# Autodesk Inventor assembly: Assembly
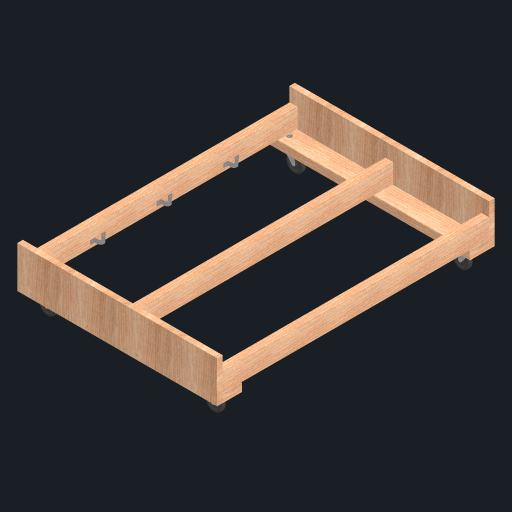
[picture p0: Inventor's stored thumbnail of the model, 512x512]
Saved by Autodesk Inventor 2024.2 (Build 282272000, 272)
## iProperties
Created: 2025-06-28
Part Number: Assembly
Document SubType Name: Assembly
Designer: Bryan
Mass: 15499.4 g
Surface Area: 23116.4 cm^2
Volume: 27379.6 cm^3
Density: 0.566091 g/cm^3
Author: Bryan
## Documents named in this file (14)
- C:\Users\bobsb\OneDrive\Documents\GitHub\PlateRack_Robotics\Assembly.iam
- C:\Users\bobsb\OneDrive\Documents\GitHub\PlateRack_Robotics\2834T25_Threaded-Stem Swivel Caster.ipt
- C:\Users\bobsb\OneDrive\Documents\GitHub\PlateRack_Robotics\Horizontal Beam 3ft.ipt
- C:\Users\bobsb\OneDrive\Documents\GitHub\PlateRack_Robotics\Horizontal Beam 4ft.ipt
- C:\Users\bobsb\OneDrive\Documents\GitHub\PlateRack_Robotics\91903A032_Medium-Strength Steel Extra-Wide Hex Nut.ipt
- C:\Users\bobsb\OneDrive\Documents\GitHub\PlateRack_Robotics\Side Panel.ipt
- C:\Users\bobsb\OneDrive\Documents\GitHub\PlateRack_Robotics\9439T44_Routing Clamp.ipt
- C:\Users\bobsb\OneDrive\Documents\GitHub\PlateRack_Robotics\90031A580_Phillips Flat Head Screws for Wood.ipt
- C:\Users\bobsb\OneDrive\Documents\GitHub\PlateRack_Robotics\Assembly\AIP\FEA\f3xuib2qo.fins
- C:\Users\bobsb\OneDrive\Documents\GitHub\PlateRack_Robotics\Assembly\AIP\FEA\f3xuib2qo.fsat
- C:\Users\bobsb\OneDrive\Documents\GitHub\PlateRack_Robotics\Assembly\AIP\FEA\f3xuib2qo.ftes
- C:\Users\bobsb\OneDrive\Documents\GitHub\PlateRack_Robotics\Assembly\AIP\FEA\f3xuib2qo.fwiz
- C:\Users\bobsb\OneDrive\Documents\GitHub\PlateRack_Robotics\Assembly\AIP\FEA\f3xuib2w0.fmsh
- C:\Users\bobsb\OneDrive\Documents\GitHub\PlateRack_Robotics\Assembly\AIP\FEA\f3xuib2w1.fres
## Components (77 placed, 7 different names)
1. 2834T25_Threaded-Stem Swivel Caster:1 — Mate:1, Mate:2, Angle:1, Mate:6
2. Horizontal Beam 3ft:1 — Mate:1, Mate:2, Angle:1, Mate:3, Mate:4, Angle:2, Flush:1, Mate:5, Flush:2, Mate:7, Mate:8, Mate:9, Flush:3, Flush:4, Flush:5, Mate:12, Mate:22, Flush:8, Mate:55, Flush:25, Mate:56, Flush:26, Mate:57, Flush:27
3. Horizontal Beam 4ft:1 — Flush:1, Mate:5, Flush:2, Mate:10, Flush:6, Flush:7, Flush:9, Flush:11, Mate:33, Mate:34, Mate:35, Mate:36, Mate:37, Mate:38, Mate:39, Mate:40, Mate:41
4. 2834T25_Threaded-Stem Swivel Caster:2 — Mate:3, Mate:4, Angle:2, Mate:11
5. 91903A032_Medium-Strength Steel Extra-Wide Hex Nut:1 — Mate:6, Mate:7
6. Horizontal Beam 4ft:2 — Mate:9, Flush:3, Flush:4, Mate:24, Mate:25, Mate:26, Mate:27, Mate:28, Mate:29, Mate:30, Mate:31, Mate:32
7. Horizontal Beam 4ft:3 — Mate:8, Flush:5, Mate:10, Mate:21
8. 91903A032_Medium-Strength Steel Extra-Wide Hex Nut:2 — Mate:11, Mate:12
9. 2834T25_Threaded-Stem Swivel Caster:3
10. Horizontal Beam 3ft:2 — Mate:21, Flush:6, Flush:7, Flush:10, Mate:23, Mate:52, Flush:22, Mate:53, Flush:23, Mate:54, Flush:24
11. 2834T25_Threaded-Stem Swivel Caster:4
12. 91903A032_Medium-Strength Steel Extra-Wide Hex Nut:3
13. 91903A032_Medium-Strength Steel Extra-Wide Hex Nut:4
14. Side Panel:1 — Mate:22, Flush:8, Flush:9, Mate:42, Flush:12, Mate:43, Flush:13, Mate:44, Flush:14, Mate:45, Flush:15, Mate:46, Flush:16
15. Side Panel:2 — Flush:10, Flush:11, Mate:23, Mate:47, Flush:17, Mate:48, Flush:18, Mate:49, Flush:19, Mate:50, Flush:20, Mate:51, Flush:21
16. 9439T44_Routing Clamp:1 — Mate:24, Mate:25, Mate:26
17. 9439T44_Routing Clamp:2 — Mate:27, Mate:28, Mate:29
18. 9439T44_Routing Clamp:3 — Mate:30, Mate:31, Mate:32
19. 9439T44_Routing Clamp:4 — Mate:33, Mate:40, Mate:41
20. 9439T44_Routing Clamp:5 — Mate:34, Mate:38, Mate:39
21. 9439T44_Routing Clamp:6 — Mate:35, Mate:36, Mate:37
22. 90031A580_Phillips Flat Head Screws for Wood:1 — Mate:42, Flush:12
23. 90031A580_Phillips Flat Head Screws for Wood:18 — Mate:45, Flush:15
24. 90031A580_Phillips Flat Head Screws for Wood:19 — Mate:46, Flush:16
25. 90031A580_Phillips Flat Head Screws for Wood:20 — Mate:47, Flush:17
26. 90031A580_Phillips Flat Head Screws for Wood:21 — Mate:48, Flush:18
27. 90031A580_Phillips Flat Head Screws for Wood:22 — Mate:49, Flush:19
28. 90031A580_Phillips Flat Head Screws for Wood:2 — Mate:43, Flush:13
29. 90031A580_Phillips Flat Head Screws for Wood:3
30. 90031A580_Phillips Flat Head Screws for Wood:4
31. 90031A580_Phillips Flat Head Screws for Wood:5
32. 90031A580_Phillips Flat Head Screws for Wood:6
33. 90031A580_Phillips Flat Head Screws for Wood:7
34. 90031A580_Phillips Flat Head Screws for Wood:8
35. 90031A580_Phillips Flat Head Screws for Wood:9
36. 90031A580_Phillips Flat Head Screws for Wood:10 — Mate:44, Flush:14
37. 90031A580_Phillips Flat Head Screws for Wood:11
38. 90031A580_Phillips Flat Head Screws for Wood:12
39. 90031A580_Phillips Flat Head Screws for Wood:13
40. 90031A580_Phillips Flat Head Screws for Wood:14
41. 90031A580_Phillips Flat Head Screws for Wood:15
42. 90031A580_Phillips Flat Head Screws for Wood:16
43. 90031A580_Phillips Flat Head Screws for Wood:17
44. 90031A580_Phillips Flat Head Screws for Wood:23 — Mate:50, Flush:20
45. 90031A580_Phillips Flat Head Screws for Wood:24
46. 90031A580_Phillips Flat Head Screws for Wood:25
47. 90031A580_Phillips Flat Head Screws for Wood:26
48. 90031A580_Phillips Flat Head Screws for Wood:27
49. 90031A580_Phillips Flat Head Screws for Wood:28
50. 90031A580_Phillips Flat Head Screws for Wood:29
51. 90031A580_Phillips Flat Head Screws for Wood:30
52. 90031A580_Phillips Flat Head Screws for Wood:31 — Mate:51, Flush:21
53. 90031A580_Phillips Flat Head Screws for Wood:32
54. 90031A580_Phillips Flat Head Screws for Wood:33
55. 90031A580_Phillips Flat Head Screws for Wood:34
56. 90031A580_Phillips Flat Head Screws for Wood:35
57. 90031A580_Phillips Flat Head Screws for Wood:36
58. 90031A580_Phillips Flat Head Screws for Wood:37
59. 90031A580_Phillips Flat Head Screws for Wood:38
60. 90031A580_Phillips Flat Head Screws for Wood:41 — Mate:54, Flush:24
61. 90031A580_Phillips Flat Head Screws for Wood:39 — Mate:52, Flush:22
62. 90031A580_Phillips Flat Head Screws for Wood:40 — Mate:53, Flush:23
63. 90031A580_Phillips Flat Head Screws for Wood:42
64. 90031A580_Phillips Flat Head Screws for Wood:43
65. 90031A580_Phillips Flat Head Screws for Wood:44
66. 90031A580_Phillips Flat Head Screws for Wood:45
67. 90031A580_Phillips Flat Head Screws for Wood:46
68. 90031A580_Phillips Flat Head Screws for Wood:47
69. 90031A580_Phillips Flat Head Screws for Wood:50 — Mate:57, Flush:27
70. 90031A580_Phillips Flat Head Screws for Wood:49 — Mate:56, Flush:26
71. 90031A580_Phillips Flat Head Screws for Wood:48 — Mate:55, Flush:25
72. 90031A580_Phillips Flat Head Screws for Wood:51
73. 90031A580_Phillips Flat Head Screws for Wood:52
74. 90031A580_Phillips Flat Head Screws for Wood:53
75. 90031A580_Phillips Flat Head Screws for Wood:54
76. 90031A580_Phillips Flat Head Screws for Wood:55
77. 90031A580_Phillips Flat Head Screws for Wood:56
## Component patterns: (8 elements, first: 90031A580_Phillips Flat Head Screws for Wood:2), (8 elements, first: 90031A580_Phillips Flat Head Screws for Wood:10), (8 elements, first: 90031A580_Phillips Flat Head Screws for Wood:23), (8 elements, first: 90031A580_Phillips Flat Head Screws for Wood:31), (3 elements, first: 90031A580_Phillips Flat Head Screws for Wood:41 + 90031A580_Phillips Flat Head Screws for Wood:39 + 90031A580_Phillips Flat Head Screws for Wood:40), (3 elements, first: 90031A580_Phillips Flat Head Screws for Wood:50 + 90031A580_Phillips Flat Head Screws for Wood:49 + 90031A580_Phillips Flat Head Screws for Wood:48)
## Relationships (88: Mate 57, Flush 27, Angle 4)
- Mate:1: 2834T25_Threaded-Stem Swivel Caster:1 ↔ Horizontal Beam 3ft:1
- Mate:2: 2834T25_Threaded-Stem Swivel Caster:1 ↔ Horizontal Beam 3ft:1
- Angle:1 (0 deg): 2834T25_Threaded-Stem Swivel Caster:1 ↔ Horizontal Beam 3ft:1
- Mate:3: Horizontal Beam 3ft:1 ↔ 2834T25_Threaded-Stem Swivel Caster:2
- Mate:4: Horizontal Beam 3ft:1 ↔ 2834T25_Threaded-Stem Swivel Caster:2
- Angle:2 (0 deg): Horizontal Beam 3ft:1 ↔ 2834T25_Threaded-Stem Swivel Caster:2
- Flush:1: Horizontal Beam 3ft:1 ↔ Horizontal Beam 4ft:1
- Mate:5: Horizontal Beam 3ft:1 ↔ Horizontal Beam 4ft:1
- Flush:2: Horizontal Beam 3ft:1 ↔ Horizontal Beam 4ft:1
- Mate:6: 2834T25_Threaded-Stem Swivel Caster:1 ↔ 91903A032_Medium-Strength Steel Extra-Wide Hex Nut:1
- Mate:7: Horizontal Beam 3ft:1 ↔ 91903A032_Medium-Strength Steel Extra-Wide Hex Nut:1
- Mate:8: Horizontal Beam 3ft:1 ↔ Horizontal Beam 4ft:3
- Mate:9: Horizontal Beam 3ft:1 ↔ Horizontal Beam 4ft:2
- Flush:3: Horizontal Beam 3ft:1 ↔ Horizontal Beam 4ft:2
- Flush:4: Horizontal Beam 3ft:1 ↔ Horizontal Beam 4ft:2
- Flush:5: Horizontal Beam 3ft:1 ↔ Horizontal Beam 4ft:3
- Mate:10 (400.05 mm): Horizontal Beam 4ft:1 ↔ Horizontal Beam 4ft:3
- Mate:11: 2834T25_Threaded-Stem Swivel Caster:2 ↔ 91903A032_Medium-Strength Steel Extra-Wide Hex Nut:2
- Mate:12: Horizontal Beam 3ft:1 ↔ 91903A032_Medium-Strength Steel Extra-Wide Hex Nut:2
- [Mate]: 2834T25_Threaded-Stem Swivel Caster:3 ↔ Horizontal Beam 3ft:2
- [Mate]: 2834T25_Threaded-Stem Swivel Caster:3 ↔ Horizontal Beam 3ft:2
- [Angle] (0 deg): 2834T25_Threaded-Stem Swivel Caster:3 ↔ Horizontal Beam 3ft:2
- [Mate]: Horizontal Beam 3ft:2 ↔ 2834T25_Threaded-Stem Swivel Caster:4
- [Mate]: Horizontal Beam 3ft:2 ↔ 2834T25_Threaded-Stem Swivel Caster:4
- [Angle] (0 deg): Horizontal Beam 3ft:2 ↔ 2834T25_Threaded-Stem Swivel Caster:4
- [Mate]: 2834T25_Threaded-Stem Swivel Caster:3 ↔ 91903A032_Medium-Strength Steel Extra-Wide Hex Nut:3
- [Mate]: Horizontal Beam 3ft:2 ↔ 91903A032_Medium-Strength Steel Extra-Wide Hex Nut:3
- [Mate]: 2834T25_Threaded-Stem Swivel Caster:4 ↔ 91903A032_Medium-Strength Steel Extra-Wide Hex Nut:4
- [Mate]: Horizontal Beam 3ft:2 ↔ 91903A032_Medium-Strength Steel Extra-Wide Hex Nut:4
- Mate:21: Horizontal Beam 4ft:3 ↔ Horizontal Beam 3ft:2
- Flush:6: Horizontal Beam 4ft:1 ↔ Horizontal Beam 3ft:2
- Flush:7: Horizontal Beam 4ft:1 ↔ Horizontal Beam 3ft:2
- Mate:22: Horizontal Beam 3ft:1 ↔ Side Panel:1
- Flush:8: Horizontal Beam 3ft:1 ↔ Side Panel:1
- Flush:9: Horizontal Beam 4ft:1 ↔ Side Panel:1
- Flush:10: Horizontal Beam 3ft:2 ↔ Side Panel:2
- Flush:11: Horizontal Beam 4ft:1 ↔ Side Panel:2
- Mate:23: Horizontal Beam 3ft:2 ↔ Side Panel:2
- Mate:24: Horizontal Beam 4ft:2 ↔ 9439T44_Routing Clamp:1
- Mate:25: Horizontal Beam 4ft:2 ↔ 9439T44_Routing Clamp:1
- Mate:26: Horizontal Beam 4ft:2 ↔ 9439T44_Routing Clamp:1
- Mate:27: Horizontal Beam 4ft:2 ↔ 9439T44_Routing Clamp:2
- Mate:28: Horizontal Beam 4ft:2 ↔ 9439T44_Routing Clamp:2
- Mate:29: Horizontal Beam 4ft:2 ↔ 9439T44_Routing Clamp:2
- Mate:30: Horizontal Beam 4ft:2 ↔ 9439T44_Routing Clamp:3
- Mate:31: Horizontal Beam 4ft:2 ↔ 9439T44_Routing Clamp:3
- Mate:32: Horizontal Beam 4ft:2 ↔ 9439T44_Routing Clamp:3
- Mate:33: Horizontal Beam 4ft:1 ↔ 9439T44_Routing Clamp:4
- Mate:34: Horizontal Beam 4ft:1 ↔ 9439T44_Routing Clamp:5
- Mate:35: Horizontal Beam 4ft:1 ↔ 9439T44_Routing Clamp:6
- Mate:36: Horizontal Beam 4ft:1 ↔ 9439T44_Routing Clamp:6
- Mate:37: Horizontal Beam 4ft:1 ↔ 9439T44_Routing Clamp:6
- Mate:38: Horizontal Beam 4ft:1 ↔ 9439T44_Routing Clamp:5
- Mate:39: Horizontal Beam 4ft:1 ↔ 9439T44_Routing Clamp:5
- Mate:40: Horizontal Beam 4ft:1 ↔ 9439T44_Routing Clamp:4
- Mate:41: Horizontal Beam 4ft:1 ↔ 9439T44_Routing Clamp:4
- Mate:42: Side Panel:1 ↔ 90031A580_Phillips Flat Head Screws for Wood:1
- Flush:12: Side Panel:1 ↔ 90031A580_Phillips Flat Head Screws for Wood:1
- Mate:43: Side Panel:1 ↔ 90031A580_Phillips Flat Head Screws for Wood:2
- Flush:13: Side Panel:1 ↔ 90031A580_Phillips Flat Head Screws for Wood:2
- Mate:44: Side Panel:1 ↔ 90031A580_Phillips Flat Head Screws for Wood:10
- Flush:14: Side Panel:1 ↔ 90031A580_Phillips Flat Head Screws for Wood:10
- Mate:45: Side Panel:1 ↔ 90031A580_Phillips Flat Head Screws for Wood:18
- Flush:15: Side Panel:1 ↔ 90031A580_Phillips Flat Head Screws for Wood:18
- Mate:46: Side Panel:1 ↔ 90031A580_Phillips Flat Head Screws for Wood:19
- Flush:16: Side Panel:1 ↔ 90031A580_Phillips Flat Head Screws for Wood:19
- Mate:47: Side Panel:2 ↔ 90031A580_Phillips Flat Head Screws for Wood:20
- Flush:17: Side Panel:2 ↔ 90031A580_Phillips Flat Head Screws for Wood:20
- Mate:48: Side Panel:2 ↔ 90031A580_Phillips Flat Head Screws for Wood:21
- Flush:18: Side Panel:2 ↔ 90031A580_Phillips Flat Head Screws for Wood:21
- Mate:49: Side Panel:2 ↔ 90031A580_Phillips Flat Head Screws for Wood:22
- Flush:19: Side Panel:2 ↔ 90031A580_Phillips Flat Head Screws for Wood:22
- Mate:50: Side Panel:2 ↔ 90031A580_Phillips Flat Head Screws for Wood:23
- Flush:20: Side Panel:2 ↔ 90031A580_Phillips Flat Head Screws for Wood:23
- Mate:51: Side Panel:2 ↔ 90031A580_Phillips Flat Head Screws for Wood:31
- Flush:21: Side Panel:2 ↔ 90031A580_Phillips Flat Head Screws for Wood:31
- Mate:52: Horizontal Beam 3ft:2 ↔ 90031A580_Phillips Flat Head Screws for Wood:39
- Flush:22: Horizontal Beam 3ft:2 ↔ 90031A580_Phillips Flat Head Screws for Wood:39
- Mate:53: Horizontal Beam 3ft:2 ↔ 90031A580_Phillips Flat Head Screws for Wood:40
- Flush:23: Horizontal Beam 3ft:2 ↔ 90031A580_Phillips Flat Head Screws for Wood:40
- Mate:54: Horizontal Beam 3ft:2 ↔ 90031A580_Phillips Flat Head Screws for Wood:41
- Flush:24: Horizontal Beam 3ft:2 ↔ 90031A580_Phillips Flat Head Screws for Wood:41
- Mate:55: Horizontal Beam 3ft:1 ↔ 90031A580_Phillips Flat Head Screws for Wood:48
- Flush:25: Horizontal Beam 3ft:1 ↔ 90031A580_Phillips Flat Head Screws for Wood:48
- Mate:56: Horizontal Beam 3ft:1 ↔ 90031A580_Phillips Flat Head Screws for Wood:49
- Flush:26: Horizontal Beam 3ft:1 ↔ 90031A580_Phillips Flat Head Screws for Wood:49
- Mate:57: Horizontal Beam 3ft:1 ↔ 90031A580_Phillips Flat Head Screws for Wood:50
- Flush:27: Horizontal Beam 3ft:1 ↔ 90031A580_Phillips Flat Head Screws for Wood:50
## Named parameters: d19_d0 = 0 mm, d20_d1 = 0 mm, d21_d2 = 0 deg, d22_d17 = 0 mm, d23_d18 = 0 mm, d24_d3 = 0 mm, d25_d4 = 0 mm, d26_d5 = 0 deg, d27_d9 = 0 mm, d28_d10 = 0 mm, sa_0 = 3102.64
note: some values were not read from the file. Shown as the stored number, unit unknown: "sa_0".
